# Autodesk Inventor assembly: full_layout_test
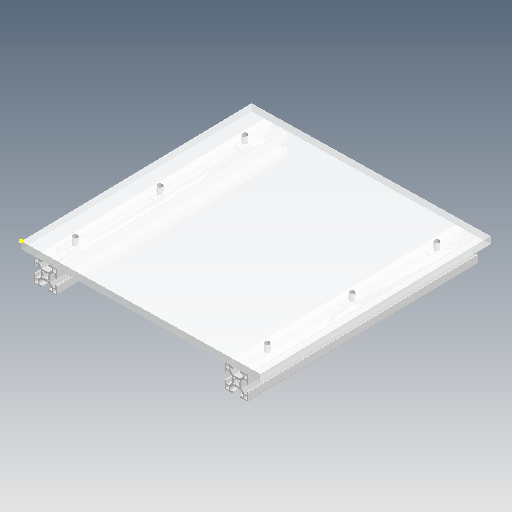
[picture p0: Inventor's stored thumbnail of the model, 512x512]
Saved by Autodesk Inventor 2025.4 (Build 294407020, 407B)
## iProperties
Created: 2026-09-08
Part Number: full_layout_test
Document SubType Name: Assembly
Designer: Aiden
Author: Aiden
## Documents named in this file (5)
- C:\Users\Aiden\Documents\GitHub\coldex-instrumentation\3d_models\mounting_hardware\dummy_parts\full_layout_test.iam
- C:\Users\Aiden\Documents\GitHub\coldex-instrumentation\3d_models\mounting_hardware\dummy_parts\acrylic_base.ipt
- C:\Users\Aiden\Documents\GitHub\coldex-instrumentation\3d_models\mounting_hardware\dummy_parts\acrylic_cover.ipt
- C:\Users\Aiden\Documents\GitHub\coldex-instrumentation\3d_models\mounting_hardware\McMaster\30mm_1ft_T-Slotted Framing.ipt
- C:\Users\Aiden\Documents\GitHub\coldex-instrumentation\3d_models\mounting_hardware\McMaster\30mm_teenut_T-Slotted Framing.ipt
## Components (10 placed, 4 different names)
1. acrylic_base:1 — Flush:1, Flush:2, Mate:1, Mate:2, Flush:3, Flush:4, Mate:9, Mate:10, Mate:11, Mate:12, Mate:13, Mate:14
2. acrylic_cover:1 — Flush:1, Flush:2
3. 30mm_1ft_T-Slotted Framing:1 — Mate:1, Flush:4, Mate:3, Mate:4, Mate:5, Tangent:2
4. 30mm_1ft_T-Slotted Framing:2 — Mate:2, Flush:3, Mate:6, Mate:7, Mate:8, Tangent:1
5. 30mm_teenut_T-Slotted Framing:1 — Mate:5, Mate:9
6. 30mm_teenut_T-Slotted Framing:2 — Mate:3, Mate:10
7. 30mm_teenut_T-Slotted Framing:3 — Mate:4, Mate:11, Tangent:2
8. 30mm_teenut_T-Slotted Framing:4 — Mate:7, Mate:13
9. 30mm_teenut_T-Slotted Framing:5 — Mate:6, Mate:14
10. 30mm_teenut_T-Slotted Framing:6 — Mate:8, Mate:12, Tangent:1
## Relationships (20: Mate 14, Flush 4, Tangent 2)
- Flush:1: acrylic_base:1 ↔ acrylic_cover:1
- Flush:2: acrylic_base:1 ↔ acrylic_cover:1
- Mate:1: acrylic_base:1 ↔ 30mm_1ft_T-Slotted Framing:1
- Mate:2: acrylic_base:1 ↔ 30mm_1ft_T-Slotted Framing:2
- Flush:3: acrylic_base:1 ↔ 30mm_1ft_T-Slotted Framing:2
- Flush:4: acrylic_base:1 ↔ 30mm_1ft_T-Slotted Framing:1
- Mate:3: 30mm_1ft_T-Slotted Framing:1 ↔ 30mm_teenut_T-Slotted Framing:2
- Mate:4: 30mm_1ft_T-Slotted Framing:1 ↔ 30mm_teenut_T-Slotted Framing:3
- Mate:5: 30mm_1ft_T-Slotted Framing:1 ↔ 30mm_teenut_T-Slotted Framing:1
- Mate:6: 30mm_1ft_T-Slotted Framing:2 ↔ 30mm_teenut_T-Slotted Framing:5
- Mate:7: 30mm_1ft_T-Slotted Framing:2 ↔ 30mm_teenut_T-Slotted Framing:4
- Mate:8: 30mm_1ft_T-Slotted Framing:2 ↔ 30mm_teenut_T-Slotted Framing:6
- Mate:9: acrylic_base:1 ↔ 30mm_teenut_T-Slotted Framing:1
- Mate:10: acrylic_base:1 ↔ 30mm_teenut_T-Slotted Framing:2
- Mate:11: acrylic_base:1 ↔ 30mm_teenut_T-Slotted Framing:3
- Mate:12: acrylic_base:1 ↔ 30mm_teenut_T-Slotted Framing:6
- Mate:13: acrylic_base:1 ↔ 30mm_teenut_T-Slotted Framing:4
- Mate:14: acrylic_base:1 ↔ 30mm_teenut_T-Slotted Framing:5
- Tangent:1: 30mm_1ft_T-Slotted Framing:2 ↔ 30mm_teenut_T-Slotted Framing:6
- Tangent:2: 30mm_1ft_T-Slotted Framing:1 ↔ 30mm_teenut_T-Slotted Framing:3
